# Autodesk Inventor assembly: Chassi 3-1-2020
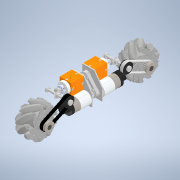
[picture p0: Inventor's stored thumbnail of the model, 180x180]
Saved by Autodesk Inventor 2020.2 (Build 242310000, 310)
## iProperties
Created: 2019-12-09
Part Number: Chassi 3-1-2020
Document SubType Name: Assembly
Designer: deli
Author: deli
## Documents named in this file (19)
- C:\Users\deli\OneDrive - Eastside Preparatory School\FTC\Chassi\Chassi 3-1-2020.iam
- C:\Users\deli\OneDrive - Eastside Preparatory School\Documents\Personal\Maslow\Side Channel.ipt
- C:\Users\deli\OneDrive - Eastside Preparatory School\FTC\Chassi\100 mm mecanum wheel.ipt
- C:\Users\deli\OneDrive - Eastside Preparatory School\FTC\Chassi\0_500_Hex_ID_x_1_125_OD_x_0_313_WD_Flanged_Bearing_v2_217-3875 v1.ipt
- C:\Users\deli\OneDrive - Eastside Preparatory School\FTC\Chassi\MecanumSideplates v1.ipt
- C:\Users\deli\OneDrive - Eastside Preparatory School\FTC\Chassi\MecanumSideplates with 18t belt gear.ipt
- C:\Users\deli\OneDrive - Eastside Preparatory School\FTC\Chassi\Axel for wheels 1_2_Hex_x_0_201_ID_ThunderHex_Stock_36_217-4017.ipt
- C:\Users\deli\OneDrive - Eastside Preparatory School\FTC\Chassi\100 mm mecanum wheel_MIR.ipt
- C:\Users\deli\OneDrive - Eastside Preparatory School\FTC\Chassi\Gearbox with neverest.iam
- C:\Users\deli\Downloads\download\615442 assembly.ipt
- C:\Users\deli\OneDrive - Eastside Preparatory School\FTC\Chassi\6mm axel from gearbox.ipt
- C:\Users\deli\OneDrive - Eastside Preparatory School\FTC\Chassi\1611-0514-0006.ipt
- C:\Users\deli\OneDrive - Eastside Preparatory School\FTC\Chassi\6mm axel for bevel gear and pully.ipt
- C:\Users\deli\OneDrive - Eastside Preparatory School\FTC\Chassi\615398 assembly.ipt
- C:\Users\deli\OneDrive - Eastside Preparatory School\FTC\Chassi\Gearbox with neverest_MIR1.iam
- C:\Users\deli\OneDrive - Eastside Preparatory School\FTC\Chassi\6mm axel from gearbox_MIR.ipt
- C:\Users\deli\OneDrive - Eastside Preparatory School\FTC\Chassi\615398 assembly_MIR.ipt
- C:\Users\deli\OneDrive - Eastside Preparatory School\FTC\Chassi\18t belt gear for bevel gear axel.ipt
- C:\Users\deli\OneDrive - Eastside Preparatory School\FTC\Chassi\49T belt from gobuilda.ipt
## Components (32 placed, 18 different names)
1. Side Channel:1 — Mate:61, Mate:62, Mate:67, Mate:68, Mate:69, Mate:70, Mate:78, Mate:79, Mate:80, Mate:81, Mate:82, Mate:83, Mate:84, Mate:85, Mate:99, Mate:100
2. 0_500_Hex_ID_x_1_125_OD_x_0_313_WD_Flanged_Bearing_v2_217-3875 v1:3 — Flush:5, Mate:67, Mate:68, Mate:106
3. 0_500_Hex_ID_x_1_125_OD_x_0_313_WD_Flanged_Bearing_v2_217-3875 v1:4
4. MecanumSideplates v1:2 — Mate:65
5. MecanumSideplates with 18t belt gear:2 — Mate:64, Mate:66
6. Axel for wheels 1_2_Hex_x_0_201_ID_ThunderHex_Stock_36_217-4017:2 — Mate:63, Flush:5
7. 100 mm mecanum wheel:3 — Rotation:4
8. 0_500_Hex_ID_x_1_125_OD_x_0_313_WD_Flanged_Bearing_v2_217-3875 v1:5 — Mate:61, Flush:4, Mate:62, Mate:109
9. 0_500_Hex_ID_x_1_125_OD_x_0_313_WD_Flanged_Bearing_v2_217-3875 v1:6
10. MecanumSideplates v1:3
11. MecanumSideplates with 18t belt gear:3
12. Axel for wheels 1_2_Hex_x_0_201_ID_ThunderHex_Stock_36_217-4017:3 — Flush:4
13. 100 mm mecanum wheel_MIR:1 — Mate:63, Mate:64, Mate:65, Mate:66, Rotation:5
14. Gearbox with neverest:1 [sub-assembly] — Mate:69, Mate:70, Mate:75, Mate:76, Mate:89, Mate:92
15. 615442 assembly:1
16. 6mm axel from gearbox:1 — Mate:75, Mate:76, Mate:88
17. 1611-0514-0006:1 — Mate:81, Mate:82, Mate:86, Flush:6
18. 1611-0514-0006:2 — Mate:80, Mate:83, Mate:87, Flush:7
19. 1611-0514-0006:3 — Mate:78, Mate:85, Mate:103
20. 1611-0514-0006:4 — Mate:79, Mate:84, Mate:105
21. 6mm axel for bevel gear and pully:1 — Mate:87, Flush:7, Mate:90, Mate:91, Mate:104, Angle:14, Rotation:3, Angle:15
22. 6mm axel for bevel gear and pully:2 — Mate:86, Flush:6, Mate:101, Mate:102, Angle:13, Angle:16
23. 615398 assembly:1 — Mate:88, Mate:89, Mate:91, Rotation:1
24. 615398 assembly:2 — Mate:90, Mate:92, Rotation:1, Rotation:3, Angle:15
25. Gearbox with neverest_MIR1:1 [sub-assembly] — Mate:93, Mate:94, Mate:95, Mate:97, Mate:99, Mate:100
26. 6mm axel from gearbox_MIR:1 — Mate:93, Mate:94, Mate:96
27. 615398 assembly_MIR:1 — Mate:95, Mate:96, Rotation:2, Mate:98
28. 615398 assembly_MIR:2 — Rotation:2, Mate:97, Mate:98, Mate:101, Angle:16
29. 18t belt gear for bevel gear axel:1 — Mate:102, Angle:13, Mate:103, Rotation:5, Mate:107
30. 18t belt gear for bevel gear axel:2 — Mate:104, Angle:14, Mate:105, Rotation:4, Mate:108
31. 49T belt from gobuilda:1 — Mate:106, Mate:107
32. 49T belt from gobuilda:2 — Mate:108, Mate:109
## Relationships (85: Mate 62, Angle 12, Flush 6, RelateRotation 5)
- [Mate]: 0_500_Hex_ID_x_1_125_OD_x_0_313_WD_Flanged_Bearing_v2_217-3875 v1:4 ↔ MecanumSideplates v1:2
- [Mate]: 0_500_Hex_ID_x_1_125_OD_x_0_313_WD_Flanged_Bearing_v2_217-3875 v1:4 ↔ Axel for wheels 1_2_Hex_x_0_201_ID_ThunderHex_Stock_36_217-4017:2
- [Angle] (0 deg): 0_500_Hex_ID_x_1_125_OD_x_0_313_WD_Flanged_Bearing_v2_217-3875 v1:4 ↔ Axel for wheels 1_2_Hex_x_0_201_ID_ThunderHex_Stock_36_217-4017:2
- [Mate]: MecanumSideplates v1:2 ↔ Axel for wheels 1_2_Hex_x_0_201_ID_ThunderHex_Stock_36_217-4017:2
- [Angle] (0 deg): MecanumSideplates v1:2 ↔ Axel for wheels 1_2_Hex_x_0_201_ID_ThunderHex_Stock_36_217-4017:2
- [Mate]: MecanumSideplates with 18t belt gear:2 ↔ Axel for wheels 1_2_Hex_x_0_201_ID_ThunderHex_Stock_36_217-4017:2
- [Angle] (0 deg): MecanumSideplates with 18t belt gear:2 ↔ Axel for wheels 1_2_Hex_x_0_201_ID_ThunderHex_Stock_36_217-4017:2
- [Mate]: 0_500_Hex_ID_x_1_125_OD_x_0_313_WD_Flanged_Bearing_v2_217-3875 v1:3 ↔ Axel for wheels 1_2_Hex_x_0_201_ID_ThunderHex_Stock_36_217-4017:2
- [Angle] (0 deg): 0_500_Hex_ID_x_1_125_OD_x_0_313_WD_Flanged_Bearing_v2_217-3875 v1:3 ↔ Axel for wheels 1_2_Hex_x_0_201_ID_ThunderHex_Stock_36_217-4017:2
- [Flush]: 0_500_Hex_ID_x_1_125_OD_x_0_313_WD_Flanged_Bearing_v2_217-3875 v1:4 ↔ Axel for wheels 1_2_Hex_x_0_201_ID_ThunderHex_Stock_36_217-4017:2
- [Mate]: 100 mm mecanum wheel:3 ↔ 0_500_Hex_ID_x_1_125_OD_x_0_313_WD_Flanged_Bearing_v2_217-3875 v1:5
- [Mate]: 100 mm mecanum wheel:3 ↔ MecanumSideplates v1:3
- [Mate]: 100 mm mecanum wheel:3 ↔ MecanumSideplates v1:3
- [Mate]: 100 mm mecanum wheel:3 ↔ MecanumSideplates v1:3
- [Mate]: 0_500_Hex_ID_x_1_125_OD_x_0_313_WD_Flanged_Bearing_v2_217-3875 v1:6 ↔ MecanumSideplates v1:3
- [Mate]: 100 mm mecanum wheel:3 ↔ MecanumSideplates with 18t belt gear:3
- [Mate]: 100 mm mecanum wheel:3 ↔ MecanumSideplates with 18t belt gear:3
- [Mate]: 100 mm mecanum wheel:3 ↔ MecanumSideplates with 18t belt gear:3
- [Mate]: 0_500_Hex_ID_x_1_125_OD_x_0_313_WD_Flanged_Bearing_v2_217-3875 v1:6 ↔ Axel for wheels 1_2_Hex_x_0_201_ID_ThunderHex_Stock_36_217-4017:3
- [Angle] (0 deg): 0_500_Hex_ID_x_1_125_OD_x_0_313_WD_Flanged_Bearing_v2_217-3875 v1:6 ↔ Axel for wheels 1_2_Hex_x_0_201_ID_ThunderHex_Stock_36_217-4017:3
- [Mate]: MecanumSideplates v1:3 ↔ Axel for wheels 1_2_Hex_x_0_201_ID_ThunderHex_Stock_36_217-4017:3
- [Angle] (0 deg): MecanumSideplates v1:3 ↔ Axel for wheels 1_2_Hex_x_0_201_ID_ThunderHex_Stock_36_217-4017:3
- [Mate]: 100 mm mecanum wheel:3 ↔ Axel for wheels 1_2_Hex_x_0_201_ID_ThunderHex_Stock_36_217-4017:3
- [Mate]: MecanumSideplates with 18t belt gear:3 ↔ Axel for wheels 1_2_Hex_x_0_201_ID_ThunderHex_Stock_36_217-4017:3
- [Angle] (0 deg): MecanumSideplates with 18t belt gear:3 ↔ Axel for wheels 1_2_Hex_x_0_201_ID_ThunderHex_Stock_36_217-4017:3
- [Mate]: 0_500_Hex_ID_x_1_125_OD_x_0_313_WD_Flanged_Bearing_v2_217-3875 v1:5 ↔ Axel for wheels 1_2_Hex_x_0_201_ID_ThunderHex_Stock_36_217-4017:3
- [Angle] (0 deg): 0_500_Hex_ID_x_1_125_OD_x_0_313_WD_Flanged_Bearing_v2_217-3875 v1:5 ↔ Axel for wheels 1_2_Hex_x_0_201_ID_ThunderHex_Stock_36_217-4017:3
- [Flush]: 0_500_Hex_ID_x_1_125_OD_x_0_313_WD_Flanged_Bearing_v2_217-3875 v1:6 ↔ Axel for wheels 1_2_Hex_x_0_201_ID_ThunderHex_Stock_36_217-4017:3
- Mate:61: Side Channel:1 ↔ 0_500_Hex_ID_x_1_125_OD_x_0_313_WD_Flanged_Bearing_v2_217-3875 v1:5
- Flush:4: 0_500_Hex_ID_x_1_125_OD_x_0_313_WD_Flanged_Bearing_v2_217-3875 v1:5 ↔ Axel for wheels 1_2_Hex_x_0_201_ID_ThunderHex_Stock_36_217-4017:3
- Mate:62: Side Channel:1 ↔ 0_500_Hex_ID_x_1_125_OD_x_0_313_WD_Flanged_Bearing_v2_217-3875 v1:5
- Mate:63: Axel for wheels 1_2_Hex_x_0_201_ID_ThunderHex_Stock_36_217-4017:2 ↔ 100 mm mecanum wheel_MIR:1
- Mate:64: MecanumSideplates with 18t belt gear:2 ↔ 100 mm mecanum wheel_MIR:1
- Mate:65: MecanumSideplates v1:2 ↔ 100 mm mecanum wheel_MIR:1
- Mate:66: MecanumSideplates with 18t belt gear:2 ↔ 100 mm mecanum wheel_MIR:1
- Flush:5: 0_500_Hex_ID_x_1_125_OD_x_0_313_WD_Flanged_Bearing_v2_217-3875 v1:3 ↔ Axel for wheels 1_2_Hex_x_0_201_ID_ThunderHex_Stock_36_217-4017:2
- Mate:67: Side Channel:1 ↔ 0_500_Hex_ID_x_1_125_OD_x_0_313_WD_Flanged_Bearing_v2_217-3875 v1:3
- Mate:68: Side Channel:1 ↔ 0_500_Hex_ID_x_1_125_OD_x_0_313_WD_Flanged_Bearing_v2_217-3875 v1:3
- Mate:69: Side Channel:1 ↔ Gearbox with neverest:1
- Mate:70: Side Channel:1 ↔ Gearbox with neverest:1
- Mate:75: Gearbox with neverest:1 ↔ 6mm axel from gearbox:1
- Mate:76: Gearbox with neverest:1 ↔ 6mm axel from gearbox:1
- Mate:78: Side Channel:1 ↔ 1611-0514-0006:3
- Mate:79: Side Channel:1 ↔ 1611-0514-0006:4
- Mate:80: Side Channel:1 ↔ 1611-0514-0006:2
- Mate:81: Side Channel:1 ↔ 1611-0514-0006:1
- Mate:82: Side Channel:1 ↔ 1611-0514-0006:1
- Mate:83: Side Channel:1 ↔ 1611-0514-0006:2
- Mate:84: Side Channel:1 ↔ 1611-0514-0006:4
- Mate:85: Side Channel:1 ↔ 1611-0514-0006:3
- Mate:86: 1611-0514-0006:1 ↔ 6mm axel for bevel gear and pully:2
- Flush:6: 1611-0514-0006:1 ↔ 6mm axel for bevel gear and pully:2
- Mate:87: 1611-0514-0006:2 ↔ 6mm axel for bevel gear and pully:1
- Flush:7: 1611-0514-0006:2 ↔ 6mm axel for bevel gear and pully:1
- Mate:88: 6mm axel from gearbox:1 ↔ 615398 assembly:1
- Mate:89: Gearbox with neverest:1 ↔ 615398 assembly:1
- Mate:90: 6mm axel for bevel gear and pully:1 ↔ 615398 assembly:2
- Mate:91 (-16.7132 mm): 6mm axel for bevel gear and pully:1 ↔ 615398 assembly:1
- Mate:92 (-16.7132 mm): Gearbox with neverest:1 ↔ 615398 assembly:2
- Rotation:1 [RelateRotation] (1 ul): 615398 assembly:1 ↔ 615398 assembly:2
- Mate:93: Gearbox with neverest_MIR1:1 ↔ 6mm axel from gearbox_MIR:1
- Mate:94: Gearbox with neverest_MIR1:1 ↔ 6mm axel from gearbox_MIR:1
- Mate:95: Gearbox with neverest_MIR1:1 ↔ 615398 assembly_MIR:1
- Mate:96: 6mm axel from gearbox_MIR:1 ↔ 615398 assembly_MIR:1
- Rotation:2 [RelateRotation] (1 ul): 615398 assembly_MIR:1 ↔ 615398 assembly_MIR:2
- Mate:97 (-16.7132 mm): Gearbox with neverest_MIR1:1 ↔ 615398 assembly_MIR:2
- Mate:98 (-16.7132 mm): 615398 assembly_MIR:1 ↔ 615398 assembly_MIR:2
- Mate:99: Side Channel:1 ↔ Gearbox with neverest_MIR1:1
- Mate:100: Side Channel:1 ↔ Gearbox with neverest_MIR1:1
- Mate:101: 6mm axel for bevel gear and pully:2 ↔ 615398 assembly_MIR:2
- Mate:102: 6mm axel for bevel gear and pully:2 ↔ 18t belt gear for bevel gear axel:1
- Angle:13 (0 deg): 6mm axel for bevel gear and pully:2 ↔ 18t belt gear for bevel gear axel:1
- Mate:103: 1611-0514-0006:3 ↔ 18t belt gear for bevel gear axel:1
- Mate:104: 6mm axel for bevel gear and pully:1 ↔ 18t belt gear for bevel gear axel:2
- Angle:14 (0 deg): 6mm axel for bevel gear and pully:1 ↔ 18t belt gear for bevel gear axel:2
- Mate:105: 1611-0514-0006:4 ↔ 18t belt gear for bevel gear axel:2
- Rotation:3 [RelateRotation] (0.482 ul): 6mm axel for bevel gear and pully:1 ↔ 615398 assembly:2
- Angle:15 (0 deg): 6mm axel for bevel gear and pully:1 ↔ 615398 assembly:2
- Rotation:4 [RelateRotation] (1 ul): 100 mm mecanum wheel:3 ↔ 18t belt gear for bevel gear axel:2
- Angle:16 (0 deg): 6mm axel for bevel gear and pully:2 ↔ 615398 assembly_MIR:2
- Rotation:5 [RelateRotation] (1 ul): 100 mm mecanum wheel_MIR:1 ↔ 18t belt gear for bevel gear axel:1
- Mate:106: 0_500_Hex_ID_x_1_125_OD_x_0_313_WD_Flanged_Bearing_v2_217-3875 v1:3 ↔ 49T belt from gobuilda:1
- Mate:107: 18t belt gear for bevel gear axel:1 ↔ 49T belt from gobuilda:1
- Mate:108: 18t belt gear for bevel gear axel:2 ↔ 49T belt from gobuilda:2
- Mate:109: 0_500_Hex_ID_x_1_125_OD_x_0_313_WD_Flanged_Bearing_v2_217-3875 v1:5 ↔ 49T belt from gobuilda:2
## Named parameters: d45_d25 = 0 mm, d49_d30 = 0 mm, d50_d31 = 0 deg, d51_d33 = 0 mm, d52_d34 = 0 deg, d54_d36 = 0 mm, d55_d37 = 0 deg, d56_d38 = 0 mm, d57_d39 = 0 deg, d58_d40 = 0 mm, d59_d7 = 0 mm, d60_d11 = 0 mm, d61_d12 = 0 mm, d62_d13 = 0 mm, d63_d25 = 0 mm, d64_d26 = 0 mm, d65_d28 = 0 mm, d66_d29 = 0 mm, d67_d30 = 0 mm, d68_d31 = 0 deg, d69_d33 = 0 mm, d70_d34 = 0 deg, d71_d35 = 0 mm, d72_d36 = 0 mm, d73_d37 = 0 deg, d74_d38 = 0 mm, d75_d39 = 0 deg, d76_d40 = 0 mm
